# Autodesk Inventor assembly: racked
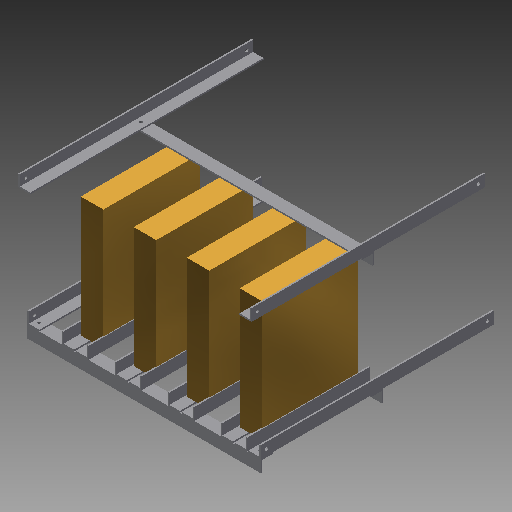
[picture p0: Inventor's stored thumbnail of the model, 512x512]
Saved by Autodesk Inventor 2017 (Build 210142000, 142)
## iProperties
Created: 2018-10-22
Part Number: racked
Document SubType Name: Assembly
Designer: ddeboer
Author: ddeboer
## Documents named in this file (4)
- C:\Users\ddeboer\Desktop\snap_holder\racked_3.iam
- C:\Users\ddeboer\Desktop\snap_holder\bottom.iam
- C:\Users\ddeboer\Desktop\snap_holder\snap.ipt
- C:\Users\ddeboer\Desktop\snap_holder\top_3.iam
## Components (6 placed, 3 different names)
1. bottom:1 [sub-assembly] — Flush:1
2. top_3:1 [sub-assembly] — Flush:1, Mate:1, Mate:2
3. snap:1 — Mate:1, Mate:2
4. snap:2
5. snap:3
6. snap:4
## Component patterns: (4 elements, first: snap:1)
## Relationships (3: Mate 2, Flush 1)
- Flush:1: bottom:1 ↔ top_3:1
- Mate:1: top_3:1 ↔ snap:1
- Mate:2: top_3:1 ↔ snap:1
